# Autodesk Inventor assembly: HbIndexFingerForChild
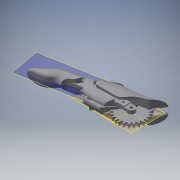
[picture p0: Inventor's stored thumbnail of the model, 180x180]
Saved by Autodesk Inventor 2017 (Build 210142000, 142)
## iProperties
Part Number: HbIndexFingerForChild
Material: 一般
Document SubType Name: Assembly
Designer: sktom
Author: sktom
## Documents named in this file (10)
- D:\OneDrive\CAD\MAJ\hackberry\HACKberry-hardware\3D_69%\Inventor\HbHandForChild\HbIndexFinger01ForChild\HbIndexFinger01ForChild.iam
- D:\OneDrive\CAD\MAJ\hackberry\HACKberry-hardware\3D_69%\Inventor\HbHandForChild\HbIndexFinger01ForChild\HbIndexInputLink02ForChild.ipt
- D:\OneDrive\CAD\MAJ\hackberry\HACKberry-hardware\3D_69%\Inventor\HbHandForChild\HbIndexFinger01ForChild\HbIndexMiddle-DistalPhalanx02ForChild.ipt
- D:\OneDrive\CAD\MAJ\hackberry\HACKberry-hardware\3D_69%\Inventor\HbHandForChild\HbIndexFinger01ForChild\HbIndexCouplerLink02ForChild.ipt
- D:\OneDrive\CAD\MAJ\hackberry\HACKberry-hardware\3D_69%\Inventor\HbHandForChild\HbIndexFinger01ForChild\HbIndexCouplerLinkCover02ForChild.ipt
- D:\OneDrive\CAD\MAJ\hackberry\HACKberry-hardware\3D_69%\Inventor\HbHandForChild\HbIndexFinger01ForChild\HbIndexProximalPhalanx03ForChild.ipt
- D:\OneDrive\CAD\MAJ\hackberry\HACKberry-hardware\3D_69%\Inventor\HbHandForChild\HbIndexFinger01ForChild\HbIndexProximalPhalanxCover02ForChild.ipt
- D:\OneDrive\CAD\MAJ\hackberry\HACKberry-hardware\3D_69%\Inventor\HbHandForChild\HbIndexFinger01ForChild\Shaft_phi2_L8.ipt
- D:\OneDrive\CAD\MAJ\hackberry\HACKberry-hardware\3D_69%\Inventor\HbHandForChild\HbIndexFinger01ForChild\M2_L8.ipt
- D:\OneDrive\CAD\MAJ\hackberry\HACKberry-hardware\3D_69%\Inventor\HbHandForChild\HbIndexFinger01ForChild\HbIndexReleaseLever02ForChild.ipt
## Components (15 placed, 9 different names)
1. HbIndexInputLink02ForChild:1 — 挿入:4, 円柱状:1
2. HbIndexMiddle-DistalPhalanx02ForChild:1 — 挿入:1, 挿入:5
3. HbIndexCouplerLink02ForChild:1 — 挿入:1, 挿入:2, 挿入:3, 挿入:4, 挿入:9
4. HbIndexCouplerLinkCover02ForChild:1 — 挿入:2, 挿入:3, 挿入:10, 挿入:11, 挿入:14
5. HbIndexProximalPhalanx03ForChild:1 — 挿入:6, 挿入:7, 挿入:12, 挿入:13
6. HbIndexProximalPhalanxCover02ForChild:1 — 挿入:5, 挿入:6, 挿入:7, 円柱状:1, 挿入:8, 挿入:17
7. Shaft_phi2_L8:1 — 挿入:8
8. Shaft_phi2_L8:2 — 挿入:9
9. M2_L8:1 — 挿入:10
10. M2_L8:2 — 挿入:11
11. M2_L8:3 — 挿入:12
12. M2_L8:4 — 挿入:13
13. Shaft_phi2_L8:3 — 挿入:14
14. HbIndexReleaseLever02ForChild:1 — 挿入:16, 挿入:17
15. Shaft_phi2_L8:4 — 挿入:16
## Relationships (17: Insert 16, CylindricalJoint 1)
- 挿入:1 [Insert] (0.4 mm): HbIndexMiddle-DistalPhalanx02ForChild:1 ↔ HbIndexCouplerLink02ForChild:1
- 挿入:2 [Insert]: HbIndexCouplerLink02ForChild:1 ↔ HbIndexCouplerLinkCover02ForChild:1
- 挿入:3 [Insert]: HbIndexCouplerLink02ForChild:1 ↔ HbIndexCouplerLinkCover02ForChild:1
- 挿入:4 [Insert] (0.25 mm): HbIndexInputLink02ForChild:1 ↔ HbIndexCouplerLink02ForChild:1
- 挿入:5 [Insert] (0.4 mm): HbIndexMiddle-DistalPhalanx02ForChild:1 ↔ HbIndexProximalPhalanxCover02ForChild:1
- 挿入:6 [Insert]: HbIndexProximalPhalanx03ForChild:1 ↔ HbIndexProximalPhalanxCover02ForChild:1
- 挿入:7 [Insert]: HbIndexProximalPhalanx03ForChild:1 ↔ HbIndexProximalPhalanxCover02ForChild:1
- 円柱状:1 [CylindricalJoint]: HbIndexInputLink02ForChild:1 ↔ HbIndexProximalPhalanxCover02ForChild:1
- 挿入:8 [Insert] (0.5 mm): HbIndexProximalPhalanxCover02ForChild:1 ↔ Shaft_phi2_L8:1
- 挿入:9 [Insert] (0.5 mm): HbIndexCouplerLink02ForChild:1 ↔ Shaft_phi2_L8:2
- 挿入:10 [Insert]: HbIndexCouplerLinkCover02ForChild:1 ↔ M2_L8:1
- 挿入:11 [Insert]: HbIndexCouplerLinkCover02ForChild:1 ↔ M2_L8:2
- 挿入:12 [Insert]: HbIndexProximalPhalanx03ForChild:1 ↔ M2_L8:3
- 挿入:13 [Insert]: HbIndexProximalPhalanx03ForChild:1 ↔ M2_L8:4
- 挿入:14 [Insert] (-2.5 mm): HbIndexCouplerLinkCover02ForChild:1 ↔ Shaft_phi2_L8:3
- 挿入:16 [Insert] (-2.5 mm): HbIndexReleaseLever02ForChild:1 ↔ Shaft_phi2_L8:4
- 挿入:17 [Insert] (0.2 mm): HbIndexProximalPhalanxCover02ForChild:1 ↔ HbIndexReleaseLever02ForChild:1
